# Autodesk Inventor assembly: Assembly2
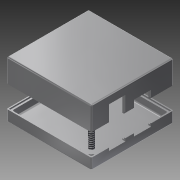
[picture p0: Inventor's stored thumbnail of the model, 180x180]
Saved by Autodesk Inventor 2013 (Build 170138000, 138)
## iProperties
Created: 2013-03-06
Part Number: Assembly2
Document SubType Name: Assembly
Designer: md
Author: md
## Documents named in this file (5)
- X:\Projects\hexasense\enclosure\power_board\Assembly2.iam
- X:\Projects\hexasense\enclosure\power_board\Oberschale2.ipt
- X:\PROJECTS\HEXASENSE\ENCLOSURE\POWER_BOARD\PCB-Model.ipt
- X:\PROJECTS\HEXASENSE\ENCLOSURE\POWER_BOARD\Unterschale2.ipt
- C:\Users\md\Documents\Inventor\Content Center Files\R2013\en-US\ISO 7049 - C-Z(2)\ISO 7049 - ST 3,5 x 22 - C - Z.ipt
## Components (5 placed, 4 different names)
1. Oberschale2:1 — Insert:5, Insert:6, Mate:3
2. PCB-Model:1 — Insert:3, Insert:4, Mate:1, Mate:2
3. Unterschale2:1 — Insert:1, Insert:2, Mate:1, Mate:2, Mate:3
4. ISO 7049 - C-Z ST 3,5 x 22 - C - Z:1 — Insert:1, Insert:4, Insert:6
5. ISO 7049 - C-Z ST 3,5 x 22 - C - Z:2 — Insert:2, Insert:3, Insert:5
## Relationships (9: Insert 6, Mate 3)
- Insert:3: PCB-Model:1 ↔ ISO 7049 - C-Z ST 3,5 x 22 - C - Z:2
- Insert:4: PCB-Model:1 ↔ ISO 7049 - C-Z ST 3,5 x 22 - C - Z:1
- Mate:1: PCB-Model:1 ↔ Unterschale2:1
- Mate:2: PCB-Model:1 ↔ Unterschale2:1
- Insert:5: Oberschale2:1 ↔ ISO 7049 - C-Z ST 3,5 x 22 - C - Z:2
- Insert:6: Oberschale2:1 ↔ ISO 7049 - C-Z ST 3,5 x 22 - C - Z:1
- Mate:3: Oberschale2:1 ↔ Unterschale2:1
- Insert:1: Unterschale2:1 ↔ ISO 7049 - C-Z ST 3,5 x 22 - C - Z:1
- Insert:2: Unterschale2:1 ↔ ISO 7049 - C-Z ST 3,5 x 22 - C - Z:2
